# Autodesk Inventor assembly: Motor Assembly
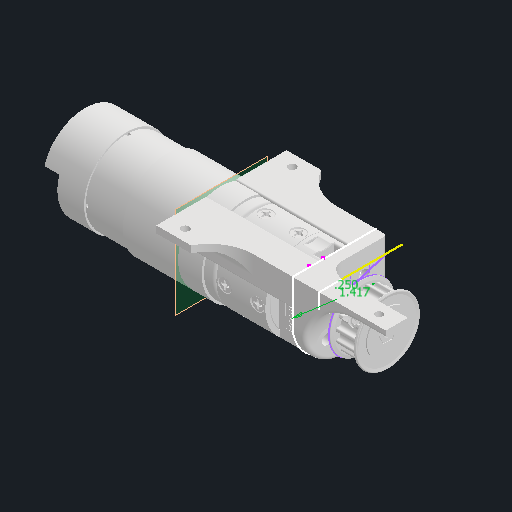
[picture p0: Inventor's stored thumbnail of the model, 512x512]
Saved by Autodesk Inventor 2022 (Build 260153000, 153)
## iProperties
Created: 2021-11-02
Part Number: Motor Assembly
Document SubType Name: Assembly
Designer: divid
Author: divid
## Documents named in this file (4)
- C:\Users\divid\Documents\GitHub\ComputerAidedDesign\2021-22\FTC\#13822 Robovikes\Drivetrain\Motor Assembly.iam
- C:\Users\divid\Documents\GitHub\ComputerAidedDesign\2021-22\FTC\#13822 Robovikes\Drivetrain\Yellow Jacket Motor\5203 Series Yellow Jacket Planetary Gear Motor (3.7 to 1 Ratio, 24mm Length 8mm REX Shaft, 1620 RPM, 3.3 - 5V Encoder) 5203-2402-000.iam
- C:\Users\divid\Documents\GitHub\ComputerAidedDesign\2021-22\FTC\#13822 Robovikes\Drivetrain\Custom GoBilda Yellow Jacket Motor Mount.ipt
- C:\Users\divid\Documents\GitHub\ComputerAidedDesign\2021-22\FTC\Parts\GoBilda\3414 Series 5mm HTD Pitch Set Screw Pinion Timing Belt Pulley (8mm REX Bore, 16 Tooth) 3414-4008-0016.iam
## Components (3 placed, 3 different names)
1. 5203 Series Yellow Jacket Planetary Gear Motor (3.7 to 1 Ratio, 24mm Length 8mm REX Shaft, 1620 RPM, 3.3 - 5V Encoder) 5203-2402-000:1 [sub-assembly]
2. Custom GoBilda Yellow Jacket Motor Mount:1
3. 3414 Series 5mm HTD Pitch Set Screw Pinion Timing Belt Pulley (8mm REX Bore, 16 Tooth) 3414-4008-0016:1 [sub-assembly]
## Relationships (6: Mate 5, Flush 1)
- [Mate]: 5203 Series Yellow Jacket Planetary Gear Motor (3.7 to 1 Ratio, 24mm Length 8mm REX Shaft, 1620 RPM, 3.3 - 5V Encoder) 5203-2402-000:1 ↔ Custom GoBilda Yellow Jacket Motor Mount:1
- [Mate]: 5203 Series Yellow Jacket Planetary Gear Motor (3.7 to 1 Ratio, 24mm Length 8mm REX Shaft, 1620 RPM, 3.3 - 5V Encoder) 5203-2402-000:1 ↔ Custom GoBilda Yellow Jacket Motor Mount:1
- [Mate]: 5203 Series Yellow Jacket Planetary Gear Motor (3.7 to 1 Ratio, 24mm Length 8mm REX Shaft, 1620 RPM, 3.3 - 5V Encoder) 5203-2402-000:1 ↔ Custom GoBilda Yellow Jacket Motor Mount:1
- [Mate]: 5203 Series Yellow Jacket Planetary Gear Motor (3.7 to 1 Ratio, 24mm Length 8mm REX Shaft, 1620 RPM, 3.3 - 5V Encoder) 5203-2402-000:1 ↔ 3414 Series 5mm HTD Pitch Set Screw Pinion Timing Belt Pulley (8mm REX Bore, 16 Tooth) 3414-4008-0016:1
- [Mate]: 5203 Series Yellow Jacket Planetary Gear Motor (3.7 to 1 Ratio, 24mm Length 8mm REX Shaft, 1620 RPM, 3.3 - 5V Encoder) 5203-2402-000:1 ↔ 3414 Series 5mm HTD Pitch Set Screw Pinion Timing Belt Pulley (8mm REX Bore, 16 Tooth) 3414-4008-0016:1
- [Flush]: 5203 Series Yellow Jacket Planetary Gear Motor (3.7 to 1 Ratio, 24mm Length 8mm REX Shaft, 1620 RPM, 3.3 - 5V Encoder) 5203-2402-000:1 ↔ 3414 Series 5mm HTD Pitch Set Screw Pinion Timing Belt Pulley (8mm REX Bore, 16 Tooth) 3414-4008-0016:1
